# Autodesk Inventor assembly: robotAssemble
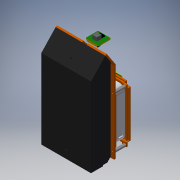
[picture p0: Inventor's stored thumbnail of the model, 180x180]
Saved by Autodesk Inventor 2019 (Build 230136000, 136)
## iProperties
Created: 2019-02-11
Part Number: robotAssemble
Document SubType Name: Assembly
Designer: izsoandras
Author: izsoandras
## Documents named in this file (9)
- D:\Users\Tarsoly\Dokumentumok\BME\6. félév\Önlab\Váz\robotAssemble.iam
- D:\Users\Tarsoly\Dokumentumok\BME\6. félév\Önlab\Váz\kocsi.ipt
- D:\Users\Tarsoly\Dokumentumok\BME\6. félév\Önlab\Váz\Wemos.ipt
- D:\Users\Tarsoly\Dokumentumok\BME\6. félév\Önlab\Váz\Yoobao.ipt
- D:\Users\Tarsoly\Dokumentumok\BME\6. félév\Önlab\Váz\RasPI.ipt
- D:\Users\Tarsoly\Dokumentumok\BME\6. félév\Önlab\Váz\RasPIcam.ipt
- D:\Users\Tarsoly\Dokumentumok\BME\6. félév\Önlab\Váz\akksi-raspi.ipt
- D:\Users\Tarsoly\Dokumentumok\BME\6. félév\Önlab\Váz\RasPItavt.ipt
- D:\Users\Tarsoly\Dokumentumok\BME\6. félév\Önlab\Váz\chassis-akksi.ipt
## Components (11 placed, 8 different names)
1. kocsi:1 — Mate:1, Mate:2, Flush:1, Flush:2
2. Wemos:1 — Mate:1, Mate:2, Flush:1, Mate:3, Flush:11, Flush:12
3. Yoobao:1 — Mate:3, Flush:2, Mate:12
4. RasPIcam:1 — Flush:13, Mate:15, Flush:14
5. akksi-raspi:1 — Mate:4, Flush:5, Mate:5, Mate:6, Mate:7, Mate:8, Flush:6, Mate:9, Flush:7, Mate:10, Flush:8, Mate:11, Flush:9, Flush:10, Mate:14
6. RasPItavt:1 — Mate:6, Flush:8, Mate:11
7. RasPItavt:2 — Mate:8, Flush:6, Mate:9
8. RasPItavt:3 — Mate:7, Flush:7, Mate:10
9. RasPItavt:4 — Mate:4, Flush:5, Mate:5, Mate:13
10. RasPI:1 — Flush:9, Flush:10, Mate:14, Flush:13
11. chassis-akksi:1 — Flush:11, Mate:12, Mate:13, Flush:12, Mate:15, Flush:14
## Relationships (27: Mate 15, Flush 12)
- Mate:1 (7 mm): kocsi:1 ↔ Wemos:1
- Mate:2 (10 mm): kocsi:1 ↔ Wemos:1
- Flush:1 (1 mm): kocsi:1 ↔ Wemos:1
- Mate:3 (-9 mm): Wemos:1 ↔ Yoobao:1
- Flush:2 (5.805 mm): kocsi:1 ↔ Yoobao:1
- Mate:4: akksi-raspi:1 ↔ RasPItavt:4
- Flush:5: akksi-raspi:1 ↔ RasPItavt:4
- Mate:5: akksi-raspi:1 ↔ RasPItavt:4
- Mate:6: akksi-raspi:1 ↔ RasPItavt:1
- Mate:7: akksi-raspi:1 ↔ RasPItavt:3
- Mate:8: akksi-raspi:1 ↔ RasPItavt:2
- Flush:6: akksi-raspi:1 ↔ RasPItavt:2
- Mate:9: akksi-raspi:1 ↔ RasPItavt:2
- Flush:7: akksi-raspi:1 ↔ RasPItavt:3
- Mate:10: akksi-raspi:1 ↔ RasPItavt:3
- Flush:8: akksi-raspi:1 ↔ RasPItavt:1
- Mate:11: akksi-raspi:1 ↔ RasPItavt:1
- Flush:9 (19.5 mm): akksi-raspi:1 ↔ RasPI:1
- Flush:10: akksi-raspi:1 ↔ RasPI:1
- Flush:11: Wemos:1 ↔ chassis-akksi:1
- Mate:12: Yoobao:1 ↔ chassis-akksi:1
- Mate:13: RasPItavt:4 ↔ chassis-akksi:1
- Mate:14 (2 mm): akksi-raspi:1 ↔ RasPI:1
- Flush:12: Wemos:1 ↔ chassis-akksi:1
- Flush:13 (-2.39 mm): RasPIcam:1 ↔ RasPI:1
- Mate:15 (20 mm): RasPIcam:1 ↔ chassis-akksi:1
- Flush:14 (-41 mm): RasPIcam:1 ↔ chassis-akksi:1
